# Autodesk Inventor assembly: DoorAssembly
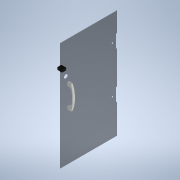
[picture p0: Inventor's stored thumbnail of the model, 180x180]
Saved by Autodesk Inventor 2021.3 (Build 253353000, 353)
## iProperties
Created: 2021-05-13
Part Number: DoorAssembly
Document SubType Name: Assembly
Designer: gisen
Author: gisen
## Documents named in this file (4)
- C:\Users\gisen\GitProjects\CAD-Data\CuboidAccessories\SecurityBox\Assemblies\DoorAssembly.iam
- C:\Users\gisen\GitProjects\CAD-Data\CuboidAccessories\SecurityBox\3DPrintedParts\DoorLockHook.ipt
- C:\Users\gisen\GitProjects\CAD-Data\CuboidAccessories\SecurityBox\Plates\DoorPlateLower.ipt
- C:\Users\gisen\GitProjects\CAD-Data\GeneralComponentsTemplate\Handles\ArkHandle-AHPF.ipt
## Components (3 placed, 3 different names)
1. DoorLockHook:1 — メイト:10, メイト:11, メイト:15
2. DoorPlateLower:1 — メイト:7, メイト:8, メイト:9, メイト:10, メイト:11, メイト:13, フラッシュ:1, メイト:14, メイト:15
3. ArkHandle-AHPF:1 — メイト:13, フラッシュ:1, メイト:14
## Relationships (9: Mate 8, Flush 1)
- メイト:7 [Mate]: DoorPlateLower:1
- メイト:8 [Mate]: DoorPlateLower:1
- メイト:9 [Mate]: DoorPlateLower:1
- メイト:10 [Mate]: DoorLockHook:1 ↔ DoorPlateLower:1
- メイト:11 [Mate]: DoorLockHook:1 ↔ DoorPlateLower:1
- メイト:13 [Mate]: DoorPlateLower:1 ↔ ArkHandle-AHPF:1
- フラッシュ:1 [Flush] (40 mm): DoorPlateLower:1 ↔ ArkHandle-AHPF:1
- メイト:14 [Mate]: DoorPlateLower:1 ↔ ArkHandle-AHPF:1
- メイト:15 [Mate]: DoorLockHook:1 ↔ DoorPlateLower:1
